# Autodesk Inventor assembly: FullField-ver4-1111-2021
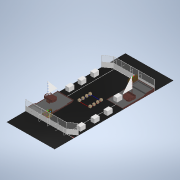
[picture p0: Inventor's stored thumbnail of the model, 180x180]
Saved by Autodesk Inventor 2021 (Build 250183000, 183)
## iProperties
Created: 2021-02-23
Part Number: FullField-ver4-1111-2021
Document SubType Name: Assembly
Designer: CMurray
Author: CMurray
## Documents named in this file (18)
- F:\PHRC CADD 2021\2021 Game Design Challenge\Full Field\Final Assembly\FullField-ver4-1111-2021.iam
- F:\PHRC CADD 2021\2021 Game Design Challenge\Full Field\Parts\FieldFloor-ver1-1111-2021.ipt
- F:\PHRC CADD 2021\2021 Game Design Challenge\Full Field\Parts\Tape\Tape.ipt
- F:\PHRC CADD 2021\2021 Game Design Challenge\Full Field\Parts\Tape\RedAllianceTape-ver1-1111-2021.ipt
- F:\PHRC CADD 2021\2021 Game Design Challenge\Full Field\Parts\Tape\BlueAllianceTape-ver1-1111-2021.ipt
- F:\PHRC CADD 2021\2021 Game Design Challenge\Player Station\Assemblies\DriverStation-ver2-1111-2021.iam
- F:\PHRC CADD 2021\2021 Game Design Challenge\Crow's Nest\Assemblies\CrowsNestFinal-ver3-1111-2021.iam
- F:\PHRC CADD 2021\2021 Game Design Challenge\Misc\MockRobot-ver1-1111-2021.ipt
- F:\PHRC CADD 2021\2021 Game Design Challenge\Main Ship\RedShip-ver1-1111-2021.ipt
- F:\PHRC CADD 2021\2021 Game Design Challenge\Crow's Nest\Parts\Capstan\test.ipt
- F:\PHRC CADD 2021\2021 Game Design Challenge\Crow's Nest\Parts\Capstan\CapTop-ver1-1111-2021.ipt
- F:\PHRC CADD 2021\2021 Game Design Challenge\Crow's Nest\Parts\Capstan\FullSailCapstan-ver2-1111-2021.iam
- F:\PHRC CADD 2021\2021 Game Design Challenge\Treasure Chest\TreasureChestFinal.ipt
- F:\PHRC CADD 2021\2021 Game Design Challenge\Full Field\Parts\Tape\Tape2.ipt
- F:\PHRC CADD 2021\2021 Game Design Challenge\Main Ship\BlueShip-ver1-1111-2021.ipt
- F:\PHRC CADD 2021\2021 Game Design Challenge\Crow's Nest\Assemblies\BlueCrowsNestFinal-ver1-1111-2021.iam
- F:\PHRC CADD 2021\2021 Game Design Challenge\Misc\cargoPrototype.ipt
- F:\PHRC CADD 2021\2021 Game Design Challenge\Full Field\Parts\Tape\MidSquareFull.iam
## Components (40 placed, 17 different names)
1. FieldFloor-ver1-1111-2021:1 — Flush:1, Flush:2, Mate:1, Mate:3, Mate:10, Flush:10, Mate:14, Flush:12, Mate:32, Mate:34, Mate:51, Flush:24, Mate:53, Flush:25, Mate:63, Mate:64, Mate:69, Mate:70, Mate:71, Mate:75, Mate:76
2. FieldFloor-ver1-1111-2021:2 — Flush:1, Flush:2, Mate:1, Mate:2, Flush:3, Flush:4, Flush:5, Flush:6, Mate:8, Flush:9, Mate:12, Flush:11, Flush:19, Mate:36, Flush:20, Mate:49, Flush:23, Mate:62, Mate:66, Mate:67, Mate:68, Mate:72, Mate:77, Mate:78, Mate:79, Mate:80, Mate:85
3. TreasureChestFinal:2 — Mate:83, Mate:84, Mate:85
4. MidSquareFull:1 [sub-assembly] — Mate:72, Mate:73, Mate:74
5. Tape2:1 — Mate:49, Flush:23, Mate:50
6. Tape2:2 — Mate:51, Flush:24, Mate:52, Mate:73
7. Tape:1 — Mate:2, Flush:3, Flush:4, Mate:9, Mate:11, Mate:33, Mate:50, Mate:74, Mate:82
8. Tape:2 — Mate:3, Flush:5, Flush:6, Mate:13, Mate:15, Mate:35, Mate:52, Mate:84
9. RedAllianceTape-ver1-1111-2021:1 — Mate:8, Flush:9, Mate:9
10. RedAllianceTape-ver1-1111-2021:2 — Mate:10, Flush:10, Mate:11
11. BlueAllianceTape-ver1-1111-2021:1 — Mate:12, Flush:11, Mate:13
12. BlueAllianceTape-ver1-1111-2021:2 — Mate:14, Flush:12, Mate:15
13. CapTop-ver1-1111-2021:2
14. FullSailCapstan-ver2-1111-2021:3 [sub-assembly] — Rotational:4
15. test:2 — Mate:57, Mate:58, Mate:59, Rotational:4
16. BlueShip-ver1-1111-2021:1 — Mate:53, Mate:54, Flush:25, Mate:55, Mate:56, Mate:65
17. BlueCrowsNestFinal-ver1-1111-2021:1 [sub-assembly] — Mate:55, Mate:56, Mate:57, Mate:58, Mate:59
18. CapTop-ver1-1111-2021:1 — Rotational:2
19. FullSailCapstan-ver2-1111-2021:2 [sub-assembly] — Rotational:1, Rotational:2
20. test:1 — Mate:41, Flush:21, Mate:42, Rotational:1
21. RedShip-ver1-1111-2021:1 — Mate:36, Mate:37, Flush:20, Mate:38, Mate:40, Mate:81, Mate:83
22. CrowsNestFinal-ver3-1111-2021:1 [sub-assembly] — Mate:38, Mate:40, Mate:41, Flush:21, Mate:42
23. DriverStation-ver2-1111-2021:2 [sub-assembly] — Mate:34, Mate:35, Flush:19, Mate:37
24. DriverStation-ver2-1111-2021:1 [sub-assembly] — Mate:32, Mate:33, Mate:54
25. cargoPrototype:2 — Mate:63
26. cargoPrototype:3 — Mate:75
27. cargoPrototype:4 — Mate:76
28. cargoPrototype:5 — Mate:78
29. cargoPrototype:6 — Mate:77
30. cargoPrototype:7 — Mate:79
31. cargoPrototype:8 — Mate:80
32. cargoPrototype:1 — Mate:62
33. TreasureChestFinal:1 — Mate:64, Mate:65, Mate:82
34. MockRobot-ver1-1111-2021:8 — Mate:81
35. MockRobot-ver1-1111-2021:1 — Mate:66
36. MockRobot-ver1-1111-2021:3 — Mate:67
37. MockRobot-ver1-1111-2021:4 — Mate:68
38. MockRobot-ver1-1111-2021:5 — Mate:69
39. MockRobot-ver1-1111-2021:6 — Mate:70
40. MockRobot-ver1-1111-2021:7 — Mate:71
## Relationships (76: Mate 56, Flush 16, RevoluteJoint 4)
- Flush:1: FieldFloor-ver1-1111-2021:1 ↔ FieldFloor-ver1-1111-2021:2
- Flush:2: FieldFloor-ver1-1111-2021:1 ↔ FieldFloor-ver1-1111-2021:2
- Mate:1: FieldFloor-ver1-1111-2021:1 ↔ FieldFloor-ver1-1111-2021:2
- Mate:2: FieldFloor-ver1-1111-2021:2 ↔ Tape:1
- Flush:3: FieldFloor-ver1-1111-2021:2 ↔ Tape:1
- Flush:4 (3606.8 mm): FieldFloor-ver1-1111-2021:2 ↔ Tape:1
- Mate:3: FieldFloor-ver1-1111-2021:1 ↔ Tape:2
- Flush:5: FieldFloor-ver1-1111-2021:2 ↔ Tape:2
- Flush:6 (3606.8 mm): FieldFloor-ver1-1111-2021:2 ↔ Tape:2
- Mate:8: FieldFloor-ver1-1111-2021:2 ↔ RedAllianceTape-ver1-1111-2021:1
- Flush:9: FieldFloor-ver1-1111-2021:2 ↔ RedAllianceTape-ver1-1111-2021:1
- Mate:9: Tape:1 ↔ RedAllianceTape-ver1-1111-2021:1
- Mate:10: FieldFloor-ver1-1111-2021:1 ↔ RedAllianceTape-ver1-1111-2021:2
- Flush:10: FieldFloor-ver1-1111-2021:1 ↔ RedAllianceTape-ver1-1111-2021:2
- Mate:11: Tape:1 ↔ RedAllianceTape-ver1-1111-2021:2
- Mate:12: FieldFloor-ver1-1111-2021:2 ↔ BlueAllianceTape-ver1-1111-2021:1
- Flush:11: FieldFloor-ver1-1111-2021:2 ↔ BlueAllianceTape-ver1-1111-2021:1
- Mate:13: Tape:2 ↔ BlueAllianceTape-ver1-1111-2021:1
- Mate:14: FieldFloor-ver1-1111-2021:1 ↔ BlueAllianceTape-ver1-1111-2021:2
- Flush:12: FieldFloor-ver1-1111-2021:1 ↔ BlueAllianceTape-ver1-1111-2021:2
- Mate:15: Tape:2 ↔ BlueAllianceTape-ver1-1111-2021:2
- Mate:32: FieldFloor-ver1-1111-2021:1 ↔ DriverStation-ver2-1111-2021:1
- Mate:33: Tape:1 ↔ DriverStation-ver2-1111-2021:1
- Mate:34: FieldFloor-ver1-1111-2021:1 ↔ DriverStation-ver2-1111-2021:2
- Mate:35: Tape:2 ↔ DriverStation-ver2-1111-2021:2
- Flush:19: FieldFloor-ver1-1111-2021:2 ↔ DriverStation-ver2-1111-2021:2
- Mate:36: FieldFloor-ver1-1111-2021:2 ↔ RedShip-ver1-1111-2021:1
- Mate:37: RedShip-ver1-1111-2021:1 ↔ DriverStation-ver2-1111-2021:2
- Flush:20: FieldFloor-ver1-1111-2021:2 ↔ RedShip-ver1-1111-2021:1
- Mate:38: RedShip-ver1-1111-2021:1 ↔ CrowsNestFinal-ver3-1111-2021:1
- Mate:40 (1778 mm): RedShip-ver1-1111-2021:1 ↔ CrowsNestFinal-ver3-1111-2021:1
- Mate:41: test:1 ↔ CrowsNestFinal-ver3-1111-2021:1
- Flush:21 (-203.2 mm): test:1 ↔ CrowsNestFinal-ver3-1111-2021:1
- Mate:42 (762 mm): test:1 ↔ CrowsNestFinal-ver3-1111-2021:1
- Rotational:1 [RevoluteJoint]: FullSailCapstan-ver2-1111-2021:2 ↔ test:1
- Rotational:2 [RevoluteJoint]: CapTop-ver1-1111-2021:1 ↔ FullSailCapstan-ver2-1111-2021:2
- Mate:49: FieldFloor-ver1-1111-2021:2 ↔ Tape2:1
- Flush:23 (1524 mm): FieldFloor-ver1-1111-2021:2 ↔ Tape2:1
- Mate:50: Tape2:1 ↔ Tape:1
- Mate:51: FieldFloor-ver1-1111-2021:1 ↔ Tape2:2
- Flush:24 (1524 mm): FieldFloor-ver1-1111-2021:1 ↔ Tape2:2
- Mate:52: Tape2:2 ↔ Tape:2
- Mate:53: FieldFloor-ver1-1111-2021:1 ↔ BlueShip-ver1-1111-2021:1
- Mate:54: BlueShip-ver1-1111-2021:1 ↔ DriverStation-ver2-1111-2021:1
- Flush:25: FieldFloor-ver1-1111-2021:1 ↔ BlueShip-ver1-1111-2021:1
- Mate:55: BlueShip-ver1-1111-2021:1 ↔ BlueCrowsNestFinal-ver1-1111-2021:1
- Mate:56 (1778 mm): BlueShip-ver1-1111-2021:1 ↔ BlueCrowsNestFinal-ver1-1111-2021:1
- Mate:57: test:2 ↔ BlueCrowsNestFinal-ver1-1111-2021:1
- Mate:58 (-203.2 mm): test:2 ↔ BlueCrowsNestFinal-ver1-1111-2021:1
- Mate:59 (762 mm): test:2 ↔ BlueCrowsNestFinal-ver1-1111-2021:1
- [RevoluteJoint]: CapTop-ver1-1111-2021:2 ↔ FullSailCapstan-ver2-1111-2021:3
- Rotational:4 [RevoluteJoint]: FullSailCapstan-ver2-1111-2021:3 ↔ test:2
- Mate:62: FieldFloor-ver1-1111-2021:2 ↔ cargoPrototype:1
- Mate:63: FieldFloor-ver1-1111-2021:1 ↔ cargoPrototype:2
- Mate:64: FieldFloor-ver1-1111-2021:1 ↔ TreasureChestFinal:1
- Mate:65: BlueShip-ver1-1111-2021:1 ↔ TreasureChestFinal:1
- Mate:66: FieldFloor-ver1-1111-2021:2 ↔ MockRobot-ver1-1111-2021:1
- Mate:67: FieldFloor-ver1-1111-2021:2 ↔ MockRobot-ver1-1111-2021:3
- Mate:68: FieldFloor-ver1-1111-2021:2 ↔ MockRobot-ver1-1111-2021:4
- Mate:69: FieldFloor-ver1-1111-2021:1 ↔ MockRobot-ver1-1111-2021:5
- Mate:70: FieldFloor-ver1-1111-2021:1 ↔ MockRobot-ver1-1111-2021:6
- Mate:71: FieldFloor-ver1-1111-2021:1 ↔ MockRobot-ver1-1111-2021:7
- Mate:72: FieldFloor-ver1-1111-2021:2 ↔ MidSquareFull:1
- Mate:73 (1930.4 mm): MidSquareFull:1 ↔ Tape2:2
- Mate:74 (6553.2 mm): MidSquareFull:1 ↔ Tape:1
- Mate:75: FieldFloor-ver1-1111-2021:1 ↔ cargoPrototype:3
- Mate:76: FieldFloor-ver1-1111-2021:1 ↔ cargoPrototype:4
- Mate:77: FieldFloor-ver1-1111-2021:2 ↔ cargoPrototype:6
- Mate:78: FieldFloor-ver1-1111-2021:2 ↔ cargoPrototype:5
- Mate:79: FieldFloor-ver1-1111-2021:2 ↔ cargoPrototype:7
- Mate:80: FieldFloor-ver1-1111-2021:2 ↔ cargoPrototype:8
- Mate:81: RedShip-ver1-1111-2021:1 ↔ MockRobot-ver1-1111-2021:8
- Mate:82: Tape:1 ↔ TreasureChestFinal:1
- Mate:83: TreasureChestFinal:2 ↔ RedShip-ver1-1111-2021:1
- Mate:84: TreasureChestFinal:2 ↔ Tape:2
- Mate:85: FieldFloor-ver1-1111-2021:2 ↔ TreasureChestFinal:2
## Named parameters: d150_d121 = 0 mm, d151_d122 = 10.074303 deg
